# Autodesk Inventor assembly: Montagem
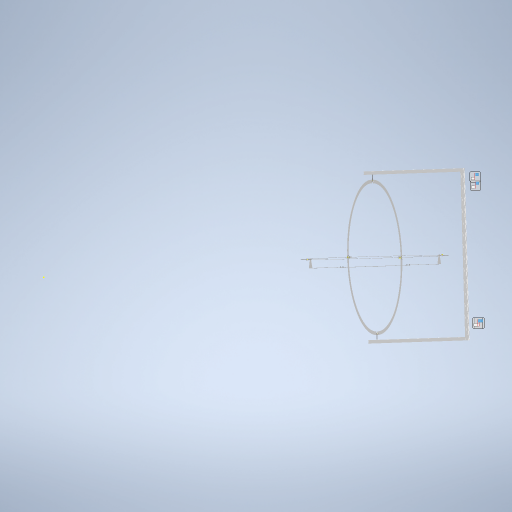
[picture p0: Inventor's stored thumbnail of the model, 512x512]
Saved by Autodesk Inventor 2024 (Build 280153000, 153)
## iProperties
Created: 2024-05-05
Part Number: Montagem
Document SubType Name: Assembly
Designer: mathe
Author: mathe
## Documents named in this file (13)
- C:\Users\mathe\OneDrive\Área de Trabalho\Plataforma de Testes\Montagem.iam
- C:\Users\mathe\OneDrive\Área de Trabalho\Plataforma de Testes\Abraçadeira.ipt
- C:\Users\mathe\OneDrive\Área de Trabalho\Plataforma de Testes\Arco menor.ipt
- C:\Users\mathe\OneDrive\Área de Trabalho\Plataforma de Testes\Arco médio.ipt
- C:\Users\mathe\OneDrive\Documentos\Inventor\Content Center Files\R2024\pt-BR\BS 4183(5)\BS 4183 - M5 x 16(2) I.ipt
- C:\Users\mathe\OneDrive\Documentos\Inventor\Content Center Files\R2024\pt-BR\ANSI B18.2.4.2M\ANSI B18.2.4.2M - M5x0,8 - 8.ipt
- C:\Users\mathe\OneDrive\Documentos\Inventor\Content Center Files\R2024\pt-BR\BS 290 SKF(19)\BS 290 SKF - SKF 108.ipt
- C:\Users\mathe\OneDrive\Documentos\Inventor\Content Center Files\R2024\pt-BR\BS EN 22 338  C - W\ISO 2338 - 8 h11 x 60 - CBS EN.ipt
- C:\Users\mathe\OneDrive\Área de Trabalho\Plataforma de Testes\Suporte Central.ipt
- C:\Users\mathe\OneDrive\Área de Trabalho\Plataforma de Testes\Suporte Drone.ipt
- C:\Users\mathe\OneDrive\Área de Trabalho\Plataforma de Testes\perfil_40x40_200 v2 com furo.ipt
- C:\Users\mathe\OneDrive\Área de Trabalho\Plataforma de Testes\perfil_40x40_200 v2.ipt
- C:\Users\mathe\OneDrive\Documentos\Inventor\Content Center Files\R2024\pt-BR\BS EN 22 338  C - W\ISO 2338 - 8 h11 x 90 - CBS EN.ipt
## Components (97 placed, 12 different names)
1. Suporte Central:1 — Coincidente:156, Coincidente:157, Coincidente:159, Ângulo:2, Coincidente:164, Coincidente:165, Coincidente:166, Coincidente:178, Coincidente:180, Coincidente:182, Coincidente:185, Ângulo:3
2. Suporte Central:2 — Coincidente:160, Coincidente:161, Coincidente:163, Ângulo:2, Coincidente:167, Coincidente:168, Coincidente:170, Coincidente:171, Coincidente:174, Coincidente:176
3. BS 290 SKF- com furo cilíndrico SKF 108:13 — Coincidente:160, Coincidente:161, Coincidente:162
4. Suporte Drone:1 — Coincidente:164, Coincidente:165, Coincidente:166, Coincidente:167, Coincidente:168, Coincidente:172, Coincidente:175, Coincidente:179, Coincidente:183
5. BS 4183 Parafuso de fenda de máquina de cabeça cilíndrica - Métrica M5 x 16:17 — Coincidente:170, Coincidente:172
6. ANSI B18.2.4.2M M5x0,8:23 — Coincidente:171
7. BS 4183 Parafuso de fenda de máquina de cabeça cilíndrica - Métrica M5 x 16:18 — Coincidente:174, Coincidente:175
8. ANSI B18.2.4.2M M5x0,8:24 — Coincidente:176
9. BS 4183 Parafuso de fenda de máquina de cabeça cilíndrica - Métrica M5 x 16:19 — Coincidente:178, Coincidente:179
10. ANSI B18.2.4.2M M5x0,8:25 — Coincidente:180
11. BS 4183 Parafuso de fenda de máquina de cabeça cilíndrica - Métrica M5 x 16:20 — Coincidente:182, Coincidente:183, Coincidente:184
12. ANSI B18.2.4.2M M5x0,8:26 — Coincidente:184, Coincidente:185
13. perfil_40x40_200 v2 com furo:1 — Coincidente:190, Coincidente:191, Ângulo:3, Coincidente:231, Coincidente:232, Ângulo:4
14. perfil_40x40_200 v2 com furo:2 — Coincidente:190, Coincidente:191, Coincidente:192, Coincidente:193
15. perfil_40x40_200 v2 com furo:3 — Coincidente:192, Coincidente:193, Coincidente:194, Coincidente:195
16. perfil_40x40_200 v2 com furo:4 — Coincidente:194, Coincidente:195, Coincidente:197, Coincidente:198
17. perfil_40x40_200 v2 com furo:5 — Coincidente:197, Coincidente:198, Coincidente:239, Coincidente:240
18. perfil_40x40_200 v2:1 — Coincidente:200, Coincidente:201
19. perfil_40x40_200 v2:2 — Coincidente:200, Coincidente:201, Coincidente:202, Coincidente:203
20. perfil_40x40_200 v2:3 — Coincidente:202, Coincidente:203, Coincidente:204, Coincidente:205
21. perfil_40x40_200 v2:4 — Coincidente:204, Coincidente:205, Coincidente:206, Coincidente:207
22. perfil_40x40_200 v2:5 — Coincidente:206, Coincidente:207, Coincidente:208, Coincidente:209
23. perfil_40x40_200 v2:6 — Coincidente:208, Coincidente:209, Coincidente:210, Coincidente:211
24. perfil_40x40_200 v2:7 — Coincidente:214, Coincidente:215, Coincidente:216, Coincidente:217
25. perfil_40x40_200 v2:8 — Coincidente:210, Coincidente:211, Coincidente:212, Coincidente:213
26. perfil_40x40_200 v2:9 — Coincidente:212, Coincidente:213, Coincidente:214, Coincidente:215
27. perfil_40x40_200 v2:10 — Coincidente:216, Coincidente:217, Coincidente:241, Coincidente:242, Ângulo:5
28. perfil_40x40_200 v2 com furo:6 — Coincidente:220, Coincidente:221, Coincidente:237, Coincidente:238
29. perfil_40x40_200 v2 com furo:7 — Coincidente:220, Coincidente:221, Coincidente:222, Coincidente:223
30. perfil_40x40_200 v2 com furo:8 — Coincidente:222, Coincidente:223, Coincidente:224, Coincidente:225
31. perfil_40x40_200 v2 com furo:9 — Coincidente:224, Coincidente:225, Coincidente:229, Coincidente:230
32. perfil_40x40_200 v2 com furo:10 — Coincidente:229, Coincidente:230, Coincidente:233, Coincidente:234, Ângulo:4
33. perfil_40x40_200 v2 com furo:11 — Coincidente:237, Coincidente:238, Coincidente:241, Coincidente:242
34. perfil_40x40_200 v2 com furo:12 — Coincidente:239, Coincidente:240
35. Abraçadeira:1 — Coincidente:1, Coincidente:2, Coincidente:3, Coincidente:4, Coincidente:31, Coincidente:44, Coincidente:47, Coincidente:67, Coincidente:68, Coincidente:71, Coincidente:92, Coincidente:99, Coincidente:100
36. Arco menor:1 — Coincidente:1, Coincidente:2, Coincidente:7, Coincidente:8
37. Arco menor:2 — Coincidente:3, Coincidente:4, Coincidente:5, Coincidente:6
38. Abraçadeira:2 — Coincidente:5, Coincidente:6, Coincidente:9, Coincidente:10, Coincidente:40, Coincidente:41, Coincidente:43, Coincidente:53, Coincidente:54, Coincidente:61, Coincidente:62, Coincidente:64, Coincidente:159
39. Abraçadeira:3 — Coincidente:7, Coincidente:8, Coincidente:59, Coincidente:60, Coincidente:84, Coincidente:85, Coincidente:86, Coincidente:87, Coincidente:103, Coincidente:104, Coincidente:154, Coincidente:163
40. Arco menor:3 — Coincidente:13, Coincidente:14
41. Arco menor:4 — Coincidente:9, Coincidente:10, Coincidente:11, Coincidente:12
42. Abraçadeira:4 — Coincidente:11, Coincidente:12, Coincidente:13, Coincidente:14, Coincidente:30, Coincidente:49, Coincidente:50, Coincidente:80, Coincidente:81, Coincidente:82, Coincidente:83, Coincidente:119, Coincidente:120, Coincidente:151
43. Arco médio:1 — Coincidente:15, Coincidente:16, Coincidente:21, Coincidente:22, Ângulo:5
44. Arco médio:2 — Coincidente:17, Coincidente:18, Coincidente:19, Coincidente:20
45. Arco médio:3 — Coincidente:25, Coincidente:26, Coincidente:27, Coincidente:28, Coincidente:29
46. Arco médio:4 — Coincidente:23, Coincidente:24
47. Abraçadeira:5 — Coincidente:15, Coincidente:16, Coincidente:17, Coincidente:18, Coincidente:31, Coincidente:45, Coincidente:48, Coincidente:65, Coincidente:66, Coincidente:69, Coincidente:70, Coincidente:94, Coincidente:96
48. Abraçadeira:6 — Coincidente:25, Coincidente:26, Coincidente:29, Coincidente:30, Coincidente:51, Coincidente:52, Coincidente:76, Coincidente:77, Coincidente:78, Coincidente:79, Coincidente:115, Coincidente:116, Coincidente:151
49. Abraçadeira:7 — Coincidente:19, Coincidente:20, Coincidente:27, Coincidente:28, Coincidente:57, Coincidente:58, Coincidente:88, Coincidente:89, Coincidente:90, Coincidente:91, Coincidente:107, Coincidente:108
50. Abraçadeira:8 — Coincidente:21, Coincidente:22, Coincidente:23, Coincidente:24, Coincidente:55, Coincidente:56, Coincidente:72, Coincidente:73, Coincidente:74, Coincidente:75, Coincidente:110, Coincidente:112
51. BS EN 22338 C - extraído 8 h11 x 60 - C:3 — Coincidente:152, Coincidente:153, Coincidente:158
52. BS EN 22338 C - extraído 8 h11 x 60 - C:4 — Coincidente:154, Coincidente:155, Coincidente:162
53. BS 290 SKF- com furo cilíndrico SKF 108:12 — Coincidente:156, Coincidente:157, Coincidente:158
54. BS 4183 Parafuso de fenda de máquina de cabeça cilíndrica - Métrica M5 x 16:1 — Coincidente:40, Coincidente:41, Coincidente:42
55. ANSI B18.2.4.2M M5x0,8:1 — Coincidente:42, Coincidente:43
56. BS 290 SKF- com furo cilíndrico SKF 108:1 — Coincidente:44, Coincidente:47, Coincidente:125
57. BS 290 SKF- com furo cilíndrico SKF 108:2 — Coincidente:45, Coincidente:48, Coincidente:126, Coincidente:141
58. BS 290 SKF- com furo cilíndrico SKF 108:4 — Coincidente:49, Coincidente:50, Coincidente:121, Coincidente:123, Coincidente:145
59. BS 290 SKF- com furo cilíndrico SKF 108:5 — Coincidente:51, Coincidente:52, Coincidente:122, Coincidente:142
60. BS 290 SKF- com furo cilíndrico SKF 108:6 — Coincidente:53, Coincidente:54, Coincidente:152, Coincidente:153
61. BS 290 SKF- com furo cilíndrico SKF 108:7 — Coincidente:55, Coincidente:56, Coincidente:235
62. BS 290 SKF- com furo cilíndrico SKF 108:8 — Coincidente:57, Coincidente:58, Coincidente:236
63. BS 290 SKF- com furo cilíndrico SKF 108:9 — Coincidente:59, Coincidente:60, Coincidente:155
64. BS 4183 Parafuso de fenda de máquina de cabeça cilíndrica - Métrica M5 x 16:2 — Coincidente:61, Coincidente:62, Coincidente:63
65. ANSI B18.2.4.2M M5x0,8:2 — Coincidente:63, Coincidente:64
66. BS 4183 Parafuso de fenda de máquina de cabeça cilíndrica - Métrica M5 x 16:3 — Coincidente:68, Coincidente:71, Coincidente:98
67. BS 4183 Parafuso de fenda de máquina de cabeça cilíndrica - Métrica M5 x 16:4 — Coincidente:67, Coincidente:92, Coincidente:97
68. BS 4183 Parafuso de fenda de máquina de cabeça cilíndrica - Métrica M5 x 16:5 — Coincidente:80, Coincidente:83, Coincidente:117
69. BS 4183 Parafuso de fenda de máquina de cabeça cilíndrica - Métrica M5 x 16:6 — Coincidente:81, Coincidente:82, Coincidente:118
70. BS 4183 Parafuso de fenda de máquina de cabeça cilíndrica - Métrica M5 x 16:7 — Coincidente:76, Coincidente:77, Coincidente:113
71. BS 4183 Parafuso de fenda de máquina de cabeça cilíndrica - Métrica M5 x 16:8 — Coincidente:78, Coincidente:79, Coincidente:114
72. BS 4183 Parafuso de fenda de máquina de cabeça cilíndrica - Métrica M5 x 16:9 — Coincidente:88, Coincidente:89, Coincidente:105
73. BS 4183 Parafuso de fenda de máquina de cabeça cilíndrica - Métrica M5 x 16:10 — Coincidente:90, Coincidente:91, Coincidente:106
74. BS 4183 Parafuso de fenda de máquina de cabeça cilíndrica - Métrica M5 x 16:11 — Coincidente:85, Coincidente:87, Coincidente:102
75. BS 4183 Parafuso de fenda de máquina de cabeça cilíndrica - Métrica M5 x 16:12 — Coincidente:84, Coincidente:86, Coincidente:101
76. BS 4183 Parafuso de fenda de máquina de cabeça cilíndrica - Métrica M5 x 16:13 — Coincidente:72, Coincidente:74, Coincidente:111
77. BS 4183 Parafuso de fenda de máquina de cabeça cilíndrica - Métrica M5 x 16:14 — Coincidente:73, Coincidente:75, Coincidente:109
78. ANSI B18.2.4.2M M5x0,8:3 — Coincidente:105, Coincidente:107
79. ANSI B18.2.4.2M M5x0,8:4 — Coincidente:106, Coincidente:108
80. ANSI B18.2.4.2M M5x0,8:9 — Coincidente:101, Coincidente:104
81. ANSI B18.2.4.2M M5x0,8:10 — Coincidente:102, Coincidente:103
82. ANSI B18.2.4.2M M5x0,8:11 — Coincidente:98, Coincidente:99
83. ANSI B18.2.4.2M M5x0,8:12 — Coincidente:97, Coincidente:100
84. ANSI B18.2.4.2M M5x0,8:15 — Coincidente:95, Coincidente:96
85. ANSI B18.2.4.2M M5x0,8:16 — Coincidente:93, Coincidente:94
86. BS 4183 Parafuso de fenda de máquina de cabeça cilíndrica - Métrica M5 x 16:15 — Coincidente:65, Coincidente:69, Coincidente:95
87. BS 4183 Parafuso de fenda de máquina de cabeça cilíndrica - Métrica M5 x 16:16 — Coincidente:66, Coincidente:70, Coincidente:93
88. ANSI B18.2.4.2M M5x0,8:17 — Coincidente:109, Coincidente:110
89. ANSI B18.2.4.2M M5x0,8:18 — Coincidente:111, Coincidente:112
90. ANSI B18.2.4.2M M5x0,8:19 — Coincidente:113, Coincidente:115
91. ANSI B18.2.4.2M M5x0,8:20 — Coincidente:114, Coincidente:116
92. ANSI B18.2.4.2M M5x0,8:21 — Coincidente:118, Coincidente:119
93. ANSI B18.2.4.2M M5x0,8:22 — Coincidente:117, Coincidente:120
94. BS EN 22338 C - extraído 8 h11 x 60 - C:2 — Coincidente:121, Coincidente:122, Coincidente:123, Coincidente:142, Coincidente:145
95. BS EN 22338 C - extraído 8 h11 x 60 - C:1 — Coincidente:125, Coincidente:126, Coincidente:141
96. BS EN 22338 C - extraído 8 h11 x 90 - C:1 — Coincidente:233, Coincidente:234, Coincidente:235
97. BS EN 22338 C - extraído 8 h11 x 90 - C:2 — Coincidente:231, Coincidente:232, Coincidente:236
## Relationships (204: Mate 200, Angle 4)
- Coincidente:1 [Mate]: Abraçadeira:1 ↔ Arco menor:1
- Coincidente:2 [Mate]: Abraçadeira:1 ↔ Arco menor:1
- Coincidente:3 [Mate]: Abraçadeira:1 ↔ Arco menor:2
- Coincidente:4 [Mate]: Abraçadeira:1 ↔ Arco menor:2
- Coincidente:5 [Mate]: Arco menor:2 ↔ Abraçadeira:2
- Coincidente:6 [Mate]: Arco menor:2 ↔ Abraçadeira:2
- Coincidente:7 [Mate]: Arco menor:1 ↔ Abraçadeira:3
- Coincidente:8 [Mate]: Arco menor:1 ↔ Abraçadeira:3
- Coincidente:9 [Mate]: Abraçadeira:2 ↔ Arco menor:4
- Coincidente:10 [Mate]: Abraçadeira:2 ↔ Arco menor:4
- Coincidente:11 [Mate]: Arco menor:4 ↔ Abraçadeira:4
- Coincidente:12 [Mate]: Arco menor:4 ↔ Abraçadeira:4
- Coincidente:13 [Mate]: Arco menor:3 ↔ Abraçadeira:4
- Coincidente:14 [Mate]: Arco menor:3 ↔ Abraçadeira:4
- Coincidente:15 [Mate]: Arco médio:1 ↔ Abraçadeira:5
- Coincidente:16 [Mate]: Arco médio:1 ↔ Abraçadeira:5
- Coincidente:17 [Mate]: Arco médio:2 ↔ Abraçadeira:5
- Coincidente:18 [Mate]: Arco médio:2 ↔ Abraçadeira:5
- Coincidente:19 [Mate]: Arco médio:2 ↔ Abraçadeira:7
- Coincidente:20 [Mate]: Arco médio:2 ↔ Abraçadeira:7
- Coincidente:21 [Mate]: Arco médio:1 ↔ Abraçadeira:8
- Coincidente:22 [Mate]: Arco médio:1 ↔ Abraçadeira:8
- Coincidente:23 [Mate]: Arco médio:4 ↔ Abraçadeira:8
- Coincidente:24 [Mate]: Arco médio:4 ↔ Abraçadeira:8
- Coincidente:25 [Mate]: Arco médio:3 ↔ Abraçadeira:6
- Coincidente:26 [Mate]: Arco médio:3 ↔ Abraçadeira:6
- Coincidente:27 [Mate]: Arco médio:3 ↔ Abraçadeira:7
- Coincidente:28 [Mate]: Arco médio:3 ↔ Abraçadeira:7
- Coincidente:29 [Mate]: Arco médio:3 ↔ Abraçadeira:6
- Coincidente:30 [Mate]: Abraçadeira:4 ↔ Abraçadeira:6
- Coincidente:31 [Mate]: Abraçadeira:1 ↔ Abraçadeira:5
- Coincidente:40 [Mate]: Abraçadeira:2 ↔ BS 4183 Parafuso de fenda de máquina de cabeça cilíndrica - Métrica M5 x 16:1
- Coincidente:41 [Mate]: Abraçadeira:2 ↔ BS 4183 Parafuso de fenda de máquina de cabeça cilíndrica - Métrica M5 x 16:1
- Coincidente:42 [Mate]: BS 4183 Parafuso de fenda de máquina de cabeça cilíndrica - Métrica M5 x 16:1 ↔ ANSI B18.2.4.2M M5x0,8:1
- Coincidente:43 [Mate]: Abraçadeira:2 ↔ ANSI B18.2.4.2M M5x0,8:1
- Coincidente:44 [Mate]: Abraçadeira:1 ↔ BS 290 SKF- com furo cilíndrico SKF 108:1
- Coincidente:45 [Mate]: Abraçadeira:5 ↔ BS 290 SKF- com furo cilíndrico SKF 108:2
- Coincidente:47 [Mate]: Abraçadeira:1 ↔ BS 290 SKF- com furo cilíndrico SKF 108:1
- Coincidente:48 [Mate]: Abraçadeira:5 ↔ BS 290 SKF- com furo cilíndrico SKF 108:2
- Coincidente:49 [Mate]: Abraçadeira:4 ↔ BS 290 SKF- com furo cilíndrico SKF 108:4
- Coincidente:50 [Mate]: Abraçadeira:4 ↔ BS 290 SKF- com furo cilíndrico SKF 108:4
- Coincidente:51 [Mate]: Abraçadeira:6 ↔ BS 290 SKF- com furo cilíndrico SKF 108:5
- Coincidente:52 [Mate]: Abraçadeira:6 ↔ BS 290 SKF- com furo cilíndrico SKF 108:5
- Coincidente:53 [Mate]: Abraçadeira:2 ↔ BS 290 SKF- com furo cilíndrico SKF 108:6
- Coincidente:54 [Mate]: Abraçadeira:2 ↔ BS 290 SKF- com furo cilíndrico SKF 108:6
- Coincidente:55 [Mate]: Abraçadeira:8 ↔ BS 290 SKF- com furo cilíndrico SKF 108:7
- Coincidente:56 [Mate]: Abraçadeira:8 ↔ BS 290 SKF- com furo cilíndrico SKF 108:7
- Coincidente:57 [Mate]: Abraçadeira:7 ↔ BS 290 SKF- com furo cilíndrico SKF 108:8
- Coincidente:58 [Mate]: Abraçadeira:7 ↔ BS 290 SKF- com furo cilíndrico SKF 108:8
- Coincidente:59 [Mate]: Abraçadeira:3 ↔ BS 290 SKF- com furo cilíndrico SKF 108:9
- Coincidente:60 [Mate]: Abraçadeira:3 ↔ BS 290 SKF- com furo cilíndrico SKF 108:9
- Coincidente:61 [Mate]: Abraçadeira:2 ↔ BS 4183 Parafuso de fenda de máquina de cabeça cilíndrica - Métrica M5 x 16:2
- Coincidente:62 [Mate]: Abraçadeira:2 ↔ BS 4183 Parafuso de fenda de máquina de cabeça cilíndrica - Métrica M5 x 16:2
- Coincidente:63 [Mate]: BS 4183 Parafuso de fenda de máquina de cabeça cilíndrica - Métrica M5 x 16:2 ↔ ANSI B18.2.4.2M M5x0,8:2
- Coincidente:64 [Mate]: Abraçadeira:2 ↔ ANSI B18.2.4.2M M5x0,8:2
- Coincidente:65 [Mate]: Abraçadeira:5 ↔ BS 4183 Parafuso de fenda de máquina de cabeça cilíndrica - Métrica M5 x 16:15
- Coincidente:66 [Mate]: Abraçadeira:5 ↔ BS 4183 Parafuso de fenda de máquina de cabeça cilíndrica - Métrica M5 x 16:16
- Coincidente:67 [Mate]: Abraçadeira:1 ↔ BS 4183 Parafuso de fenda de máquina de cabeça cilíndrica - Métrica M5 x 16:4
- Coincidente:68 [Mate]: Abraçadeira:1 ↔ BS 4183 Parafuso de fenda de máquina de cabeça cilíndrica - Métrica M5 x 16:3
- Coincidente:69 [Mate]: Abraçadeira:5 ↔ BS 4183 Parafuso de fenda de máquina de cabeça cilíndrica - Métrica M5 x 16:15
- Coincidente:70 [Mate]: Abraçadeira:5 ↔ BS 4183 Parafuso de fenda de máquina de cabeça cilíndrica - Métrica M5 x 16:16
- Coincidente:71 [Mate]: Abraçadeira:1 ↔ BS 4183 Parafuso de fenda de máquina de cabeça cilíndrica - Métrica M5 x 16:3
- Coincidente:72 [Mate]: Abraçadeira:8 ↔ BS 4183 Parafuso de fenda de máquina de cabeça cilíndrica - Métrica M5 x 16:13
- Coincidente:73 [Mate]: Abraçadeira:8 ↔ BS 4183 Parafuso de fenda de máquina de cabeça cilíndrica - Métrica M5 x 16:14
- Coincidente:74 [Mate]: Abraçadeira:8 ↔ BS 4183 Parafuso de fenda de máquina de cabeça cilíndrica - Métrica M5 x 16:13
- Coincidente:75 [Mate]: Abraçadeira:8 ↔ BS 4183 Parafuso de fenda de máquina de cabeça cilíndrica - Métrica M5 x 16:14
- Coincidente:76 [Mate]: Abraçadeira:6 ↔ BS 4183 Parafuso de fenda de máquina de cabeça cilíndrica - Métrica M5 x 16:7
- Coincidente:77 [Mate]: Abraçadeira:6 ↔ BS 4183 Parafuso de fenda de máquina de cabeça cilíndrica - Métrica M5 x 16:7
- Coincidente:78 [Mate]: Abraçadeira:6 ↔ BS 4183 Parafuso de fenda de máquina de cabeça cilíndrica - Métrica M5 x 16:8
- Coincidente:79 [Mate]: Abraçadeira:6 ↔ BS 4183 Parafuso de fenda de máquina de cabeça cilíndrica - Métrica M5 x 16:8
- Coincidente:80 [Mate]: Abraçadeira:4 ↔ BS 4183 Parafuso de fenda de máquina de cabeça cilíndrica - Métrica M5 x 16:5
- Coincidente:81 [Mate]: Abraçadeira:4 ↔ BS 4183 Parafuso de fenda de máquina de cabeça cilíndrica - Métrica M5 x 16:6
- Coincidente:82 [Mate]: Abraçadeira:4 ↔ BS 4183 Parafuso de fenda de máquina de cabeça cilíndrica - Métrica M5 x 16:6
- Coincidente:83 [Mate]: Abraçadeira:4 ↔ BS 4183 Parafuso de fenda de máquina de cabeça cilíndrica - Métrica M5 x 16:5
- Coincidente:84 [Mate]: Abraçadeira:3 ↔ BS 4183 Parafuso de fenda de máquina de cabeça cilíndrica - Métrica M5 x 16:12
- Coincidente:85 [Mate]: Abraçadeira:3 ↔ BS 4183 Parafuso de fenda de máquina de cabeça cilíndrica - Métrica M5 x 16:11
- Coincidente:86 [Mate]: Abraçadeira:3 ↔ BS 4183 Parafuso de fenda de máquina de cabeça cilíndrica - Métrica M5 x 16:12
- Coincidente:87 [Mate]: Abraçadeira:3 ↔ BS 4183 Parafuso de fenda de máquina de cabeça cilíndrica - Métrica M5 x 16:11
- Coincidente:88 [Mate]: Abraçadeira:7 ↔ BS 4183 Parafuso de fenda de máquina de cabeça cilíndrica - Métrica M5 x 16:9
- Coincidente:89 [Mate]: Abraçadeira:7 ↔ BS 4183 Parafuso de fenda de máquina de cabeça cilíndrica - Métrica M5 x 16:9
- Coincidente:90 [Mate]: Abraçadeira:7 ↔ BS 4183 Parafuso de fenda de máquina de cabeça cilíndrica - Métrica M5 x 16:10
- Coincidente:91 [Mate]: Abraçadeira:7 ↔ BS 4183 Parafuso de fenda de máquina de cabeça cilíndrica - Métrica M5 x 16:10
- Coincidente:92 [Mate]: Abraçadeira:1 ↔ BS 4183 Parafuso de fenda de máquina de cabeça cilíndrica - Métrica M5 x 16:4
- Coincidente:93 [Mate]: ANSI B18.2.4.2M M5x0,8:16 ↔ BS 4183 Parafuso de fenda de máquina de cabeça cilíndrica - Métrica M5 x 16:16
- Coincidente:94 [Mate]: Abraçadeira:5 ↔ ANSI B18.2.4.2M M5x0,8:16
- Coincidente:95 [Mate]: ANSI B18.2.4.2M M5x0,8:15 ↔ BS 4183 Parafuso de fenda de máquina de cabeça cilíndrica - Métrica M5 x 16:15
- Coincidente:96 [Mate]: Abraçadeira:5 ↔ ANSI B18.2.4.2M M5x0,8:15
- Coincidente:97 [Mate]: BS 4183 Parafuso de fenda de máquina de cabeça cilíndrica - Métrica M5 x 16:4 ↔ ANSI B18.2.4.2M M5x0,8:12
- Coincidente:98 [Mate]: BS 4183 Parafuso de fenda de máquina de cabeça cilíndrica - Métrica M5 x 16:3 ↔ ANSI B18.2.4.2M M5x0,8:11
- Coincidente:99 [Mate]: Abraçadeira:1 ↔ ANSI B18.2.4.2M M5x0,8:11
- Coincidente:100 [Mate]: Abraçadeira:1 ↔ ANSI B18.2.4.2M M5x0,8:12
- Coincidente:101 [Mate]: BS 4183 Parafuso de fenda de máquina de cabeça cilíndrica - Métrica M5 x 16:12 ↔ ANSI B18.2.4.2M M5x0,8:9
- Coincidente:102 [Mate]: BS 4183 Parafuso de fenda de máquina de cabeça cilíndrica - Métrica M5 x 16:11 ↔ ANSI B18.2.4.2M M5x0,8:10
- Coincidente:103 [Mate]: Abraçadeira:3 ↔ ANSI B18.2.4.2M M5x0,8:10
- Coincidente:104 [Mate]: Abraçadeira:3 ↔ ANSI B18.2.4.2M M5x0,8:9
- Coincidente:105 [Mate]: BS 4183 Parafuso de fenda de máquina de cabeça cilíndrica - Métrica M5 x 16:9 ↔ ANSI B18.2.4.2M M5x0,8:3
- Coincidente:106 [Mate]: BS 4183 Parafuso de fenda de máquina de cabeça cilíndrica - Métrica M5 x 16:10 ↔ ANSI B18.2.4.2M M5x0,8:4
- Coincidente:107 [Mate]: Abraçadeira:7 ↔ ANSI B18.2.4.2M M5x0,8:3
- Coincidente:108 [Mate]: Abraçadeira:7 ↔ ANSI B18.2.4.2M M5x0,8:4
- Coincidente:109 [Mate]: BS 4183 Parafuso de fenda de máquina de cabeça cilíndrica - Métrica M5 x 16:14 ↔ ANSI B18.2.4.2M M5x0,8:17
- Coincidente:110 [Mate]: Abraçadeira:8 ↔ ANSI B18.2.4.2M M5x0,8:17
- Coincidente:111 [Mate]: BS 4183 Parafuso de fenda de máquina de cabeça cilíndrica - Métrica M5 x 16:13 ↔ ANSI B18.2.4.2M M5x0,8:18
- Coincidente:112 [Mate]: Abraçadeira:8 ↔ ANSI B18.2.4.2M M5x0,8:18
- Coincidente:113 [Mate]: BS 4183 Parafuso de fenda de máquina de cabeça cilíndrica - Métrica M5 x 16:7 ↔ ANSI B18.2.4.2M M5x0,8:19
- Coincidente:114 [Mate]: BS 4183 Parafuso de fenda de máquina de cabeça cilíndrica - Métrica M5 x 16:8 ↔ ANSI B18.2.4.2M M5x0,8:20
- Coincidente:115 [Mate]: Abraçadeira:6 ↔ ANSI B18.2.4.2M M5x0,8:19
- Coincidente:116 [Mate]: Abraçadeira:6 ↔ ANSI B18.2.4.2M M5x0,8:20
- Coincidente:117 [Mate]: BS 4183 Parafuso de fenda de máquina de cabeça cilíndrica - Métrica M5 x 16:5 ↔ ANSI B18.2.4.2M M5x0,8:22
- Coincidente:118 [Mate]: BS 4183 Parafuso de fenda de máquina de cabeça cilíndrica - Métrica M5 x 16:6 ↔ ANSI B18.2.4.2M M5x0,8:21
- Coincidente:119 [Mate]: Abraçadeira:4 ↔ ANSI B18.2.4.2M M5x0,8:21
- Coincidente:120 [Mate]: Abraçadeira:4 ↔ ANSI B18.2.4.2M M5x0,8:22
- Coincidente:121 [Mate]: BS 290 SKF- com furo cilíndrico SKF 108:4 ↔ BS EN 22338 C - extraído 8 h11 x 60 - C:2
- Coincidente:122 [Mate]: BS 290 SKF- com furo cilíndrico SKF 108:5 ↔ BS EN 22338 C - extraído 8 h11 x 60 - C:2
- Coincidente:123 [Mate]: BS 290 SKF- com furo cilíndrico SKF 108:4 ↔ BS EN 22338 C - extraído 8 h11 x 60 - C:2
- Coincidente:125 [Mate]: BS 290 SKF- com furo cilíndrico SKF 108:1 ↔ BS EN 22338 C - extraído 8 h11 x 60 - C:1
- Coincidente:126 [Mate]: BS 290 SKF- com furo cilíndrico SKF 108:2 ↔ BS EN 22338 C - extraído 8 h11 x 60 - C:1
- Coincidente:141 [Mate]: BS 290 SKF- com furo cilíndrico SKF 108:2 ↔ BS EN 22338 C - extraído 8 h11 x 60 - C:1
- Coincidente:142 [Mate]: BS 290 SKF- com furo cilíndrico SKF 108:5 ↔ BS EN 22338 C - extraído 8 h11 x 60 - C:2
- Coincidente:145 [Mate]: BS 290 SKF- com furo cilíndrico SKF 108:4 ↔ BS EN 22338 C - extraído 8 h11 x 60 - C:2
- Coincidente:151 [Mate] (33 mm): Abraçadeira:4 ↔ Abraçadeira:6
- Coincidente:152 [Mate]: BS EN 22338 C - extraído 8 h11 x 60 - C:3 ↔ BS 290 SKF- com furo cilíndrico SKF 108:6
- Coincidente:153 [Mate]: BS EN 22338 C - extraído 8 h11 x 60 - C:3 ↔ BS 290 SKF- com furo cilíndrico SKF 108:6
- Coincidente:154 [Mate]: Abraçadeira:3 ↔ BS EN 22338 C - extraído 8 h11 x 60 - C:4
- Coincidente:155 [Mate]: BS EN 22338 C - extraído 8 h11 x 60 - C:4 ↔ BS 290 SKF- com furo cilíndrico SKF 108:9
- Coincidente:156 [Mate]: Suporte Central:1 ↔ BS 290 SKF- com furo cilíndrico SKF 108:12
- Coincidente:157 [Mate]: Suporte Central:1 ↔ BS 290 SKF- com furo cilíndrico SKF 108:12
- Coincidente:158 [Mate]: BS EN 22338 C - extraído 8 h11 x 60 - C:3 ↔ BS 290 SKF- com furo cilíndrico SKF 108:12
- Coincidente:159 [Mate] (30 mm): Suporte Central:1 ↔ Abraçadeira:2
- Coincidente:160 [Mate]: Suporte Central:2 ↔ BS 290 SKF- com furo cilíndrico SKF 108:13
- Coincidente:161 [Mate]: Suporte Central:2 ↔ BS 290 SKF- com furo cilíndrico SKF 108:13
- Coincidente:162 [Mate]: BS 290 SKF- com furo cilíndrico SKF 108:13 ↔ BS EN 22338 C - extraído 8 h11 x 60 - C:4
- Coincidente:163 [Mate] (30 mm): Suporte Central:2 ↔ Abraçadeira:3
- Ângulo:2 [Angle] (0 deg): Suporte Central:1 ↔ Suporte Central:2
- Coincidente:164 [Mate]: Suporte Central:1 ↔ Suporte Drone:1
- Coincidente:165 [Mate]: Suporte Central:1 ↔ Suporte Drone:1
- Coincidente:166 [Mate]: Suporte Central:1 ↔ Suporte Drone:1
- Coincidente:167 [Mate]: Suporte Central:2 ↔ Suporte Drone:1
- Coincidente:168 [Mate]: Suporte Central:2 ↔ Suporte Drone:1
- [Mate]: BS 4183 Parafuso de fenda de máquina de cabeça cilíndrica - Métrica M5 x 16:17 ↔ ANSI B18.2.4.2M M5x0,8:23
- Coincidente:170 [Mate]: Suporte Central:2 ↔ BS 4183 Parafuso de fenda de máquina de cabeça cilíndrica - Métrica M5 x 16:17
- Coincidente:171 [Mate]: Suporte Central:2 ↔ ANSI B18.2.4.2M M5x0,8:23
- Coincidente:172 [Mate]: Suporte Drone:1 ↔ BS 4183 Parafuso de fenda de máquina de cabeça cilíndrica - Métrica M5 x 16:17
- [Mate]: BS 4183 Parafuso de fenda de máquina de cabeça cilíndrica - Métrica M5 x 16:18 ↔ ANSI B18.2.4.2M M5x0,8:24
- Coincidente:174 [Mate]: Suporte Central:2 ↔ BS 4183 Parafuso de fenda de máquina de cabeça cilíndrica - Métrica M5 x 16:18
- Coincidente:175 [Mate]: Suporte Drone:1 ↔ BS 4183 Parafuso de fenda de máquina de cabeça cilíndrica - Métrica M5 x 16:18
- Coincidente:176 [Mate]: Suporte Central:2 ↔ ANSI B18.2.4.2M M5x0,8:24
- [Mate]: BS 4183 Parafuso de fenda de máquina de cabeça cilíndrica - Métrica M5 x 16:19 ↔ ANSI B18.2.4.2M M5x0,8:25
- Coincidente:178 [Mate]: Suporte Central:1 ↔ BS 4183 Parafuso de fenda de máquina de cabeça cilíndrica - Métrica M5 x 16:19
- Coincidente:179 [Mate]: Suporte Drone:1 ↔ BS 4183 Parafuso de fenda de máquina de cabeça cilíndrica - Métrica M5 x 16:19
- Coincidente:180 [Mate]: Suporte Central:1 ↔ ANSI B18.2.4.2M M5x0,8:25
- [Mate]: BS 4183 Parafuso de fenda de máquina de cabeça cilíndrica - Métrica M5 x 16:20 ↔ ANSI B18.2.4.2M M5x0,8:26
- Coincidente:182 [Mate]: Suporte Central:1 ↔ BS 4183 Parafuso de fenda de máquina de cabeça cilíndrica - Métrica M5 x 16:20
- Coincidente:183 [Mate]: Suporte Drone:1 ↔ BS 4183 Parafuso de fenda de máquina de cabeça cilíndrica - Métrica M5 x 16:20
- Coincidente:184 [Mate]: BS 4183 Parafuso de fenda de máquina de cabeça cilíndrica - Métrica M5 x 16:20 ↔ ANSI B18.2.4.2M M5x0,8:26
- Coincidente:185 [Mate]: Suporte Central:1 ↔ ANSI B18.2.4.2M M5x0,8:26
- Coincidente:190 [Mate]: perfil_40x40_200 v2 com furo:1 ↔ perfil_40x40_200 v2 com furo:2
- Coincidente:191 [Mate]: perfil_40x40_200 v2 com furo:1 ↔ perfil_40x40_200 v2 com furo:2
- Coincidente:192 [Mate]: perfil_40x40_200 v2 com furo:2 ↔ perfil_40x40_200 v2 com furo:3
- Coincidente:193 [Mate]: perfil_40x40_200 v2 com furo:2 ↔ perfil_40x40_200 v2 com furo:3
- Coincidente:194 [Mate]: perfil_40x40_200 v2 com furo:3 ↔ perfil_40x40_200 v2 com furo:4
- Coincidente:195 [Mate]: perfil_40x40_200 v2 com furo:3 ↔ perfil_40x40_200 v2 com furo:4
- Coincidente:197 [Mate]: perfil_40x40_200 v2 com furo:4 ↔ perfil_40x40_200 v2 com furo:5
- Coincidente:198 [Mate]: perfil_40x40_200 v2 com furo:4 ↔ perfil_40x40_200 v2 com furo:5
- Coincidente:200 [Mate]: perfil_40x40_200 v2:1 ↔ perfil_40x40_200 v2:2
- Coincidente:201 [Mate]: perfil_40x40_200 v2:1 ↔ perfil_40x40_200 v2:2
- Coincidente:202 [Mate]: perfil_40x40_200 v2:2 ↔ perfil_40x40_200 v2:3
- Coincidente:203 [Mate]: perfil_40x40_200 v2:2 ↔ perfil_40x40_200 v2:3
- Coincidente:204 [Mate]: perfil_40x40_200 v2:3 ↔ perfil_40x40_200 v2:4
- Coincidente:205 [Mate]: perfil_40x40_200 v2:3 ↔ perfil_40x40_200 v2:4
- Coincidente:206 [Mate]: perfil_40x40_200 v2:4 ↔ perfil_40x40_200 v2:5
- Coincidente:207 [Mate]: perfil_40x40_200 v2:4 ↔ perfil_40x40_200 v2:5
- Coincidente:208 [Mate]: perfil_40x40_200 v2:5 ↔ perfil_40x40_200 v2:6
- Coincidente:209 [Mate]: perfil_40x40_200 v2:5 ↔ perfil_40x40_200 v2:6
- Coincidente:210 [Mate]: perfil_40x40_200 v2:6 ↔ perfil_40x40_200 v2:8
- Coincidente:211 [Mate]: perfil_40x40_200 v2:6 ↔ perfil_40x40_200 v2:8
- Coincidente:212 [Mate]: perfil_40x40_200 v2:8 ↔ perfil_40x40_200 v2:9
- Coincidente:213 [Mate]: perfil_40x40_200 v2:8 ↔ perfil_40x40_200 v2:9
- Coincidente:214 [Mate]: perfil_40x40_200 v2:7 ↔ perfil_40x40_200 v2:9
- Coincidente:215 [Mate]: perfil_40x40_200 v2:7 ↔ perfil_40x40_200 v2:9
- Coincidente:216 [Mate]: perfil_40x40_200 v2:7 ↔ perfil_40x40_200 v2:10
- Coincidente:217 [Mate]: perfil_40x40_200 v2:7 ↔ perfil_40x40_200 v2:10
- Coincidente:220 [Mate]: perfil_40x40_200 v2 com furo:6 ↔ perfil_40x40_200 v2 com furo:7
- Coincidente:221 [Mate]: perfil_40x40_200 v2 com furo:6 ↔ perfil_40x40_200 v2 com furo:7
- Coincidente:222 [Mate]: perfil_40x40_200 v2 com furo:7 ↔ perfil_40x40_200 v2 com furo:8
- Coincidente:223 [Mate]: perfil_40x40_200 v2 com furo:7 ↔ perfil_40x40_200 v2 com furo:8
- Coincidente:224 [Mate]: perfil_40x40_200 v2 com furo:8 ↔ perfil_40x40_200 v2 com furo:9
- Coincidente:225 [Mate]: perfil_40x40_200 v2 com furo:8 ↔ perfil_40x40_200 v2 com furo:9
- Ângulo:3 [Angle] (180 deg): Suporte Central:1 ↔ perfil_40x40_200 v2 com furo:1
- Coincidente:229 [Mate]: perfil_40x40_200 v2 com furo:9 ↔ perfil_40x40_200 v2 com furo:10
- Coincidente:230 [Mate]: perfil_40x40_200 v2 com furo:9 ↔ perfil_40x40_200 v2 com furo:10
- Coincidente:231 [Mate]: perfil_40x40_200 v2 com furo:1 ↔ BS EN 22338 C - extraído 8 h11 x 90 - C:2
- Coincidente:232 [Mate]: perfil_40x40_200 v2 com furo:1 ↔ BS EN 22338 C - extraído 8 h11 x 90 - C:2
- Coincidente:233 [Mate]: perfil_40x40_200 v2 com furo:10 ↔ BS EN 22338 C - extraído 8 h11 x 90 - C:1
- Coincidente:234 [Mate]: perfil_40x40_200 v2 com furo:10 ↔ BS EN 22338 C - extraído 8 h11 x 90 - C:1
- Coincidente:235 [Mate]: BS 290 SKF- com furo cilíndrico SKF 108:7 ↔ BS EN 22338 C - extraído 8 h11 x 90 - C:1
- Coincidente:236 [Mate]: BS 290 SKF- com furo cilíndrico SKF 108:8 ↔ BS EN 22338 C - extraído 8 h11 x 90 - C:2
- Coincidente:237 [Mate]: perfil_40x40_200 v2 com furo:6 ↔ perfil_40x40_200 v2 com furo:11
- Coincidente:238 [Mate]: perfil_40x40_200 v2 com furo:6 ↔ perfil_40x40_200 v2 com furo:11
- Coincidente:239 [Mate]: perfil_40x40_200 v2 com furo:5 ↔ perfil_40x40_200 v2 com furo:12
- Coincidente:240 [Mate]: perfil_40x40_200 v2 com furo:5 ↔ perfil_40x40_200 v2 com furo:12
- Coincidente:241 [Mate]: perfil_40x40_200 v2:10 ↔ perfil_40x40_200 v2 com furo:11
- Coincidente:242 [Mate]: perfil_40x40_200 v2:10 ↔ perfil_40x40_200 v2 com furo:11
- Ângulo:4 [Angle] (0 deg): perfil_40x40_200 v2 com furo:1 ↔ perfil_40x40_200 v2 com furo:10
- Ângulo:5 [Angle] (0 deg): perfil_40x40_200 v2:10 ↔ Arco médio:1
## Named parameters: d208_d115 = 0 mm, d212_d208_d115 = 0 mm, d216_d212_d208_d115 = 0 mm, d220_d216_d212_d208_d115 = 0 mm
